# Autodesk Inventor assembly: барабан полгый 25-26
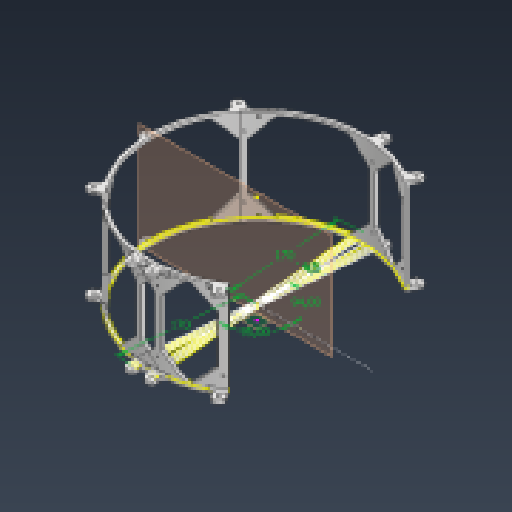
[picture p0: Inventor's stored thumbnail of the model, 512x512]
Saved by Autodesk Inventor 2026 (Build 300175000, 175)
## iProperties
Created: 2026-01-06
Part Number: барабан полгый 25-26
Document SubType Name: Assembly
Designer: Phantom
Author: Phantom
## Documents named in this file (5)
- C:\Users\GameHD\Desktop\Phantom 16950\барабан полгый 25-26.iam
- C:\Users\GameHD\Desktop\Phantom 16950\барабан для портфолио.ipt
- C:\Users\GameHD\Desktop\Phantom 16950\барабан для портфолио 2.ipt
- C:\Users\GameHD\Desktop\Phantom 16950\барабан для портфолио 3.ipt
- C:\Users\GameHD\Desktop\Phantom 16950\барабан для портфолио 2_MIR.ipt
## Components (4 placed, 4 different names)
1. барабан для портфолио:1 — Заподлицо:1, Совмещение:3, Заподлицо:2, Совмещение:4, Заподлицо:3
2. барабан для портфолио 2:1 — Совмещение:3, Заподлицо:2, Заподлицо:3
3. барабан для портфолио 3:1 — Заподлицо:1, Совмещение:4
4. барабан для портфолио 2_MIR:1
## Relationships (5: Flush 3, Mate 2)
- Заподлицо:1 [Flush]: барабан для портфолио:1 ↔ барабан для портфолио 3:1
- Совмещение:3 [Mate]: барабан для портфолио:1 ↔ барабан для портфолио 2:1
- Заподлицо:2 [Flush]: барабан для портфолио:1 ↔ барабан для портфолио 2:1
- Совмещение:4 [Mate]: барабан для портфолио:1 ↔ барабан для портфолио 3:1
- Заподлицо:3 [Flush]: барабан для портфолио:1 ↔ барабан для портфолио 2:1
